# Autodesk Inventor assembly: ASY PRS 2 Filter column D1200 940
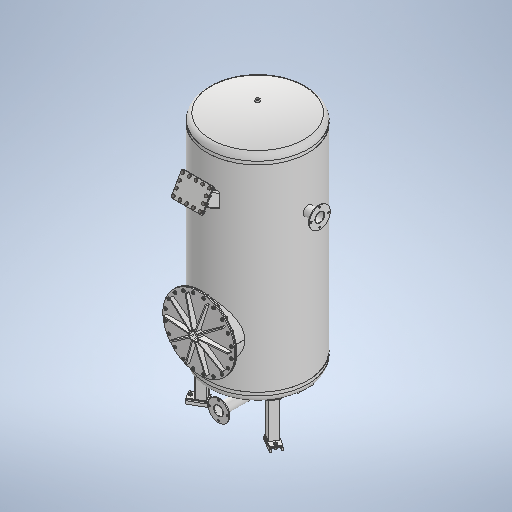
[picture p0: Inventor's stored thumbnail of the model, 512x512]
Saved by Autodesk Inventor 2026.2 (Build 302298000, 298)
## iProperties
Created: 2025-02-13
Part Number: ASY PRS 2 Filter column D1200 940
Document SubType Name: Assembly
Designer: admin
Mass: 296006 g
Surface Area: 199460 cm^2
Volume: 66339.5 cm^3
Density: 4.46198 g/cm^3
Author: pokla
Revision Number: 3
## Documents named in this file (27)
- C:\Users\admin\Documents\Inventor\PRS-Purovsk\ASY PRS 2 Filter column D1200 940.iam
- C:\Users\admin\Documents\Inventor\PRS-Purovsk\PRS 0101 main shell D1200.ipt
- C:\Users\admin\Documents\Inventor\PRS-Purovsk\PRS 0101 main shell D1200 940.ipt
- C:\Users\admin\Documents\Inventor\PRS-Purovsk\PRS 1604 dished head_D1200 940.ipt
- C:\Users\admin\Documents\Inventor\PRS-Purovsk\Fitting G1_D1200 940.ipt
- C:\Users\admin\Documents\Inventor\PRS-Purovsk\PRS 1633 charging blind flange_D1200 940.ipt
- C:\Users\admin\Documents\Inventor\PRS-Purovsk\PRS 8123 pallet jack dummy_D1200.ipt
- C:\Users\admin\Documents\Inventor\PRS-Purovsk\ASY PRS 1610 charging hatch_D1200 940.iam
- C:\Users\admin\Documents\Inventor\PRS-Purovsk\PRS 9612 accses hatch flangeipt_D1200 940.ipt
- C:\Users\admin\Documents\Inventor\PRS-Purovsk\PRS 9607 charging flange rect_D1200 940.ipt
- C:\Users\admin\Documents\Inventor\PRS-Purovsk\PRS 9606 charging flange round_D1200 940.ipt
- C:\Users\admin\Documents\Inventor\PRS-Purovsk\PRS 9672 charging tube 2_D1200 940.ipt
- C:\Users\admin\Documents\Inventor\PRS-Purovsk\PRS 9615 FDS tube 5_D1200 940.ipt
- C:\Users\admin\Documents\Inventor\PRS-Purovsk\PRS 9612 FDS tube 2_D1200 940.ipt
- C:\Users\admin\Documents\Inventor\PRS-Purovsk\cc\JIS B 2312 90 Deg Long Elbow Steel 80A x Sch 40.ipt
- C:\Users\admin\Documents\Inventor\PRS-Purovsk\PRS 9311 accses hatch tube_D1200 940.ipt
- C:\Users\admin\Documents\Inventor\PRS-Purovsk\PRS 9432 FDS free flange DN90_D1200 940.ipt
- C:\Users\admin\Documents\Inventor\PRS-Purovsk\PRS 9431 FDS flange DN90_D1200 940.ipt
- C:\Users\admin\Documents\Inventor\PRS-Purovsk\PRS 9614 FDS tube 4_D1200 940.ipt
- C:\Users\admin\Documents\Inventor\PRS-Purovsk\PRS 9613 FDS tube 3_D1200 940.ipt
- C:\Users\admin\Documents\Inventor\PRS-Purovsk\ASY PRS 9690 Filter legs D1200 940.iam
- C:\Users\admin\Documents\Inventor\PRS-Purovsk\cc\en-US\ISO 4018\ISO 4018 - M16 x 40.ipt
- C:\Users\admin\Documents\Inventor\PRS-Purovsk\cc\en-US\ISO 7089\ISO 7089 - 16 - 140 HV(1).ipt
- C:\Users\admin\Documents\Inventor\PRS-Purovsk\cc\en-US\ISO 4032(2)\ISO 4032 - M16 - ISO.ipt
- C:\Users\admin\Documents\Inventor\PRS-Purovsk\cc\en-US\ISO 4017(1)\ISO 4017 - M16 x 35 - ISO.ipt
- C:\Users\admin\Documents\Inventor\PRS-Purovsk\cc\en-US\ISO 7090\ISO 7090 - 16 - 140 HV(1).ipt
- C:\Users\admin\Documents\Inventor\PRS-Purovsk\cc\en-US\ISO 4033(2)\ISO 4033 - M16 - ISO.ipt
## Components (127 placed, 25 different names)
1. PRS 0101 main shell D1200 940:1 — Mate:1, Flush:4, Flush:2, Tangent:1, Mate:10, Mate:9, Rigid:16, Rotational:2, Rotational:3
2. PRS 1604 dished head_D1200 940:1 — Mate:8, Rigid:20, Mate:5, Mate:147, Mate:148, Rotational:2
3. PRS 1604 dished head_D1200 940:2 — Mate:4, Rigid:15, Rotational:3
4. Fitting G1_D1200 940:1 — Rigid:15
5. PRS 1633 charging blind flange_D1200 940:1 — Rigid:67
6. PRS 8123 pallet jack dummy_D1200:1
7. PRS 1633 charging blind flange_D1200 940:2 — Rigid:18
8. PRS 1633 charging blind flange_D1200 940:3 — Rigid:78
9. ASY PRS 1610 charging hatch_D1200 940:1 [sub-assembly] — Mate:12, Mate:11, Mate:51, Mate:14, Mate:13, Mate:16, Mate:15, Mate:18, Mate:17, Mate:20, Mate:19, Mate:22, Mate:21, Mate:24, Mate:23, Mate:26, Mate:25, Mate:28, Mate:27, Mate:30, Mate:29, Mate:32, Mate:31, Mate:34, Mate:33, Mate:36, Mate:35, Mate:38, Mate:37, Mate:40, Mate:39, Mate:42, Mate:41, Mate:44, Mate:43, Mate:46, Mate:45, Mate:48, Mate:47, Mate:50, Mate:49, Mate:53, Mate:55, Mate:57, Mate:59, Mate:61, Mate:63, Mate:65, Mate:67, Mate:69, Mate:71, Mate:73, Mate:75, Mate:77, Mate:79, Mate:81, Mate:83, Mate:85, Mate:87, Mate:89, Rigid:24
10. PRS 9612 accses hatch flangeipt_D1200 940:1 — Mate:52, Mate:54, Mate:56, Mate:58, Mate:60, Mate:62, Mate:64, Mate:66, Mate:68, Mate:70, Mate:72, Mate:74, Mate:76, Mate:78, Mate:80, Mate:82, Mate:84, Mate:86, Mate:88, Mate:90, Rigid:24, Rigid:23
11. PRS 9607 charging flange rect_D1200 940:1 — Mate:92, Mate:91, Mate:119, Mate:94, Mate:93, Mate:96, Mate:95, Mate:98, Mate:97, Mate:100, Mate:99, Mate:102, Mate:101, Mate:104, Mate:103, Mate:106, Mate:105, Mate:108, Mate:107, Mate:110, Mate:109, Mate:112, Mate:111, Mate:114, Mate:113, Mate:116, Mate:115, Mate:118, Mate:117, Mate:121, Mate:123, Mate:125, Mate:127, Mate:129, Mate:131, Mate:133, Mate:135, Mate:137, Mate:139, Mate:141, Mate:143, Mate:145, Rigid:83
12. PRS 9606 charging flange round_D1200 940:1 — Tangent:1, Mate:120, Mate:122, Mate:124, Mate:126, Mate:128, Mate:130, Mate:132, Mate:134, Mate:136, Mate:138, Mate:140, Mate:142, Mate:144, Mate:146, Rigid:83, Rigid:22
13. PRS 9672 charging tube 2_D1200 940:1 — Mate:10, Mate:9, Rigid:21
14. PRS 9615 FDS tube 5_D1200 940:1 — Rigid:17, Rigid:18
15. PRS 9612 FDS tube 2_D1200 940:1 — Mate:4, Rigid:78, Rigid:62
16. JIS B 2312 90 Deg Long Elbow Steel 80A x Sch 40:1 — Rigid:62, Rigid:17
17. PRS 9311 accses hatch tube_D1200 940:1 — Rigid:23, Rigid:16
18. PRS 9432 FDS free flange DN90_D1200 940:1 — Rigid:76, Rotational:71
19. PRS 9431 FDS flange DN90_D1200 940:1 — Rigid:76
20. PRS 9614 FDS tube 4_D1200 940:1 — Rigid:20, Rotational:71, Rigid:79
21. PRS 9613 FDS tube 3_D1200 940:1 — Rigid:67, Rigid:68
22. JIS B 2312 90 Deg Long Elbow Steel 80A x Sch 40:2 — Rigid:79, Rigid:68
23. Fitting G1_D1200 940:2 — Mate:8, Mate:7, Mate:6
24. ASY PRS 9690 Filter legs D1200 940:1 [sub-assembly] — Mate:2, Flush:6, Flush:5
25. PRS 9672 charging tube 2_D1200 940:2 — Rigid:22, Rigid:21
26. ISO 4018 M16 x 40:1 — Mate:12, Mate:11
27. ISO 7089 16:1 — Mate:52, Mate:51, Insert:1
28. ISO 4032 M16:1 — Insert:1
29. ISO 4018 M16 x 40:2 — Mate:14, Mate:13
30. ISO 4018 M16 x 40:3 — Mate:16, Mate:15
31. ISO 4018 M16 x 40:4 — Mate:18, Mate:17
32. ISO 4018 M16 x 40:5 — Mate:20, Mate:19
33. ISO 4018 M16 x 40:6 — Mate:22, Mate:21
34. ISO 4018 M16 x 40:7 — Mate:24, Mate:23
35. ISO 4018 M16 x 40:8 — Mate:26, Mate:25
36. ISO 4018 M16 x 40:9 — Mate:28, Mate:27
37. ISO 4018 M16 x 40:10 — Mate:30, Mate:29
38. ISO 4018 M16 x 40:11 — Mate:32, Mate:31
39. ISO 4018 M16 x 40:12 — Mate:34, Mate:33
40. ISO 4018 M16 x 40:13 — Mate:36, Mate:35
41. ISO 4018 M16 x 40:14 — Mate:38, Mate:37
42. ISO 4018 M16 x 40:15 — Mate:40, Mate:39
43. ISO 4018 M16 x 40:16 — Mate:42, Mate:41
44. ISO 4018 M16 x 40:17 — Mate:44, Mate:43
45. ISO 4018 M16 x 40:18 — Mate:46, Mate:45
46. ISO 4018 M16 x 40:19 — Mate:48, Mate:47
47. ISO 4018 M16 x 40:20 — Mate:50, Mate:49
48. ISO 7089 16:2 — Mate:54, Mate:53, Insert:2
49. ISO 7089 16:3 — Mate:56, Mate:55, Insert:3
50. ISO 7089 16:4 — Mate:58, Mate:57, Insert:4
51. ISO 7089 16:5 — Mate:60, Mate:59, Insert:5
52. ISO 7089 16:6 — Mate:62, Mate:61, Insert:6
53. ISO 7089 16:7 — Mate:64, Mate:63, Insert:7
54. ISO 7089 16:8 — Mate:66, Mate:65, Insert:8
55. ISO 7089 16:9 — Mate:68, Mate:67, Insert:9
56. ISO 7089 16:10 — Mate:70, Mate:69, Insert:10
57. ISO 7089 16:11 — Mate:72, Mate:71, Insert:11
58. ISO 7089 16:12 — Mate:74, Mate:73, Insert:12
59. ISO 7089 16:13 — Mate:76, Mate:75, Insert:13
60. ISO 7089 16:14 — Mate:78, Mate:77, Insert:14
61. ISO 7089 16:15 — Mate:80, Mate:79, Insert:15
62. ISO 7089 16:16 — Mate:82, Mate:81, Insert:16
63. ISO 7089 16:17 — Mate:84, Mate:83, Insert:17
64. ISO 7089 16:18 — Mate:86, Mate:85, Insert:18
65. ISO 7089 16:19 — Mate:88, Mate:87, Insert:19
66. ISO 7089 16:20 — Mate:90, Mate:89, Insert:20
67. ISO 4032 M16:2 — Insert:2
68. ISO 4032 M16:3 — Insert:3
69. ISO 4032 M16:4 — Insert:4
70. ISO 4032 M16:5 — Insert:5
71. ISO 4032 M16:6 — Insert:6
72. ISO 4032 M16:7 — Insert:7
73. ISO 4032 M16:8 — Insert:8
74. ISO 4032 M16:9 — Insert:9
75. ISO 4032 M16:10 — Insert:10
76. ISO 4032 M16:11 — Insert:11
77. ISO 4032 M16:12 — Insert:12
78. ISO 4032 M16:13 — Insert:13
79. ISO 4032 M16:14 — Insert:14
80. ISO 4032 M16:15 — Insert:15
81. ISO 4032 M16:16 — Insert:16
82. ISO 4032 M16:17 — Insert:17
83. ISO 4032 M16:18 — Insert:18
84. ISO 4032 M16:19 — Insert:19
85. ISO 4032 M16:20 — Insert:20
86. ISO 4017 M16 x 35:1 — Mate:92, Mate:91
87. ISO 7090 16 - 140 HV:1 — Mate:120, Mate:119, Insert:21
88. ISO 4033 M16:1 — Insert:21
89. ISO 4017 M16 x 35:2 — Mate:94, Mate:93
90. ISO 4017 M16 x 35:3 — Mate:96, Mate:95
91. ISO 4017 M16 x 35:4 — Mate:98, Mate:97
92. ISO 4017 M16 x 35:5 — Mate:100, Mate:99
93. ISO 4017 M16 x 35:6 — Mate:102, Mate:101
94. ISO 4017 M16 x 35:7 — Mate:104, Mate:103
95. ISO 4017 M16 x 35:8 — Mate:106, Mate:105
96. ISO 4017 M16 x 35:9 — Mate:108, Mate:107
97. ISO 4017 M16 x 35:10 — Mate:110, Mate:109
98. ISO 4017 M16 x 35:11 — Mate:112, Mate:111
99. ISO 4017 M16 x 35:12 — Mate:114, Mate:113
100. ISO 4017 M16 x 35:13 — Mate:116, Mate:115
101. ISO 4017 M16 x 35:14 — Mate:118, Mate:117
102. ISO 7090 16 - 140 HV:2 — Mate:122, Mate:121, Insert:22
103. ISO 7090 16 - 140 HV:3 — Mate:124, Mate:123, Insert:23
104. ISO 7090 16 - 140 HV:4 — Mate:126, Mate:125, Insert:24
105. ISO 7090 16 - 140 HV:5 — Mate:128, Mate:127, Insert:25
106. ISO 7090 16 - 140 HV:6 — Mate:130, Mate:129, Insert:26
107. ISO 7090 16 - 140 HV:7 — Mate:132, Mate:131, Insert:27
108. ISO 7090 16 - 140 HV:8 — Mate:134, Mate:133, Insert:28
109. ISO 7090 16 - 140 HV:9 — Mate:136, Mate:135, Insert:29
110. ISO 7090 16 - 140 HV:10 — Mate:138, Mate:137, Insert:30
111. ISO 7090 16 - 140 HV:11 — Mate:140, Mate:139, Insert:31
112. ISO 7090 16 - 140 HV:12 — Mate:142, Mate:141, Insert:32
113. ISO 7090 16 - 140 HV:13 — Mate:144, Mate:143, Insert:33
114. ISO 7090 16 - 140 HV:14 — Mate:146, Mate:145, Insert:34
115. ISO 4033 M16:2 — Insert:22
116. ISO 4033 M16:3 — Insert:23
117. ISO 4033 M16:4 — Insert:24
118. ISO 4033 M16:5 — Insert:25
119. ISO 4033 M16:6 — Insert:26
120. ISO 4033 M16:7 — Insert:27
121. ISO 4033 M16:8 — Insert:28
122. ISO 4033 M16:9 — Insert:29
123. ISO 4033 M16:10 — Insert:30
124. ISO 4033 M16:11 — Insert:31
125. ISO 4033 M16:12 — Insert:32
126. ISO 4033 M16:13 — Insert:33
127. ISO 4033 M16:14 — Insert:34
## Relationships (205: Mate 147, Insert 34, WeldJoint 16, Flush 4, RevoluteJoint 3, Tangent 1)
- Mate:1: PRS 0101 main shell D1200 940:1
- Flush:4: PRS 0101 main shell D1200 940:1
- Flush:2: PRS 0101 main shell D1200 940:1
- Tangent:1 (80 mm): PRS 0101 main shell D1200 940:1 ↔ PRS 9606 charging flange round_D1200 940:1
- Mate:10: PRS 0101 main shell D1200 940:1 ↔ PRS 9672 charging tube 2_D1200 940:1
- Mate:9: PRS 0101 main shell D1200 940:1 ↔ PRS 9672 charging tube 2_D1200 940:1
- Mate:4: PRS 1604 dished head_D1200 940:2 ↔ PRS 9612 FDS tube 2_D1200 940:1
- Mate:8: PRS 1604 dished head_D1200 940:1 ↔ Fitting G1_D1200 940:2
- Mate:7 (150 mm): Fitting G1_D1200 940:2
- Mate:6: Fitting G1_D1200 940:2
- Mate:2: ASY PRS 9690 Filter legs D1200 940:1
- Flush:6: ASY PRS 9690 Filter legs D1200 940:1
- Flush:5: ASY PRS 9690 Filter legs D1200 940:1
- Mate:12: ASY PRS 1610 charging hatch_D1200 940:1 ↔ ISO 4018 M16 x 40:1
- Mate:11: ASY PRS 1610 charging hatch_D1200 940:1 ↔ ISO 4018 M16 x 40:1
- Mate:52: PRS 9612 accses hatch flangeipt_D1200 940:1 ↔ ISO 7089 16:1
- Mate:51: ASY PRS 1610 charging hatch_D1200 940:1 ↔ ISO 7089 16:1
- Insert:1: ISO 7089 16:1 ↔ ISO 4032 M16:1
- Mate:14: ASY PRS 1610 charging hatch_D1200 940:1 ↔ ISO 4018 M16 x 40:2
- Mate:13: ASY PRS 1610 charging hatch_D1200 940:1 ↔ ISO 4018 M16 x 40:2
- Mate:16: ASY PRS 1610 charging hatch_D1200 940:1 ↔ ISO 4018 M16 x 40:3
- Mate:15: ASY PRS 1610 charging hatch_D1200 940:1 ↔ ISO 4018 M16 x 40:3
- Mate:18: ASY PRS 1610 charging hatch_D1200 940:1 ↔ ISO 4018 M16 x 40:4
- Mate:17: ASY PRS 1610 charging hatch_D1200 940:1 ↔ ISO 4018 M16 x 40:4
- Mate:20: ASY PRS 1610 charging hatch_D1200 940:1 ↔ ISO 4018 M16 x 40:5
- Mate:19: ASY PRS 1610 charging hatch_D1200 940:1 ↔ ISO 4018 M16 x 40:5
- Mate:22: ASY PRS 1610 charging hatch_D1200 940:1 ↔ ISO 4018 M16 x 40:6
- Mate:21: ASY PRS 1610 charging hatch_D1200 940:1 ↔ ISO 4018 M16 x 40:6
- Mate:24: ASY PRS 1610 charging hatch_D1200 940:1 ↔ ISO 4018 M16 x 40:7
- Mate:23: ASY PRS 1610 charging hatch_D1200 940:1 ↔ ISO 4018 M16 x 40:7
- Mate:26: ASY PRS 1610 charging hatch_D1200 940:1 ↔ ISO 4018 M16 x 40:8
- Mate:25: ASY PRS 1610 charging hatch_D1200 940:1 ↔ ISO 4018 M16 x 40:8
- Mate:28: ASY PRS 1610 charging hatch_D1200 940:1 ↔ ISO 4018 M16 x 40:9
- Mate:27: ASY PRS 1610 charging hatch_D1200 940:1 ↔ ISO 4018 M16 x 40:9
- Mate:30: ASY PRS 1610 charging hatch_D1200 940:1 ↔ ISO 4018 M16 x 40:10
- Mate:29: ASY PRS 1610 charging hatch_D1200 940:1 ↔ ISO 4018 M16 x 40:10
- Mate:32: ASY PRS 1610 charging hatch_D1200 940:1 ↔ ISO 4018 M16 x 40:11
- Mate:31: ASY PRS 1610 charging hatch_D1200 940:1 ↔ ISO 4018 M16 x 40:11
- Mate:34: ASY PRS 1610 charging hatch_D1200 940:1 ↔ ISO 4018 M16 x 40:12
- Mate:33: ASY PRS 1610 charging hatch_D1200 940:1 ↔ ISO 4018 M16 x 40:12
- Mate:36: ASY PRS 1610 charging hatch_D1200 940:1 ↔ ISO 4018 M16 x 40:13
- Mate:35: ASY PRS 1610 charging hatch_D1200 940:1 ↔ ISO 4018 M16 x 40:13
- Mate:38: ASY PRS 1610 charging hatch_D1200 940:1 ↔ ISO 4018 M16 x 40:14
- Mate:37: ASY PRS 1610 charging hatch_D1200 940:1 ↔ ISO 4018 M16 x 40:14
- Mate:40: ASY PRS 1610 charging hatch_D1200 940:1 ↔ ISO 4018 M16 x 40:15
- Mate:39: ASY PRS 1610 charging hatch_D1200 940:1 ↔ ISO 4018 M16 x 40:15
- Mate:42: ASY PRS 1610 charging hatch_D1200 940:1 ↔ ISO 4018 M16 x 40:16
- Mate:41: ASY PRS 1610 charging hatch_D1200 940:1 ↔ ISO 4018 M16 x 40:16
- Mate:44: ASY PRS 1610 charging hatch_D1200 940:1 ↔ ISO 4018 M16 x 40:17
- Mate:43: ASY PRS 1610 charging hatch_D1200 940:1 ↔ ISO 4018 M16 x 40:17
- Mate:46: ASY PRS 1610 charging hatch_D1200 940:1 ↔ ISO 4018 M16 x 40:18
- Mate:45: ASY PRS 1610 charging hatch_D1200 940:1 ↔ ISO 4018 M16 x 40:18
- Mate:48: ASY PRS 1610 charging hatch_D1200 940:1 ↔ ISO 4018 M16 x 40:19
- Mate:47: ASY PRS 1610 charging hatch_D1200 940:1 ↔ ISO 4018 M16 x 40:19
- Mate:50: ASY PRS 1610 charging hatch_D1200 940:1 ↔ ISO 4018 M16 x 40:20
- Mate:49: ASY PRS 1610 charging hatch_D1200 940:1 ↔ ISO 4018 M16 x 40:20
- Mate:54: PRS 9612 accses hatch flangeipt_D1200 940:1 ↔ ISO 7089 16:2
- Mate:53: ASY PRS 1610 charging hatch_D1200 940:1 ↔ ISO 7089 16:2
- Mate:56: PRS 9612 accses hatch flangeipt_D1200 940:1 ↔ ISO 7089 16:3
- Mate:55: ASY PRS 1610 charging hatch_D1200 940:1 ↔ ISO 7089 16:3
- Mate:58: PRS 9612 accses hatch flangeipt_D1200 940:1 ↔ ISO 7089 16:4
- Mate:57: ASY PRS 1610 charging hatch_D1200 940:1 ↔ ISO 7089 16:4
- Mate:60: PRS 9612 accses hatch flangeipt_D1200 940:1 ↔ ISO 7089 16:5
- Mate:59: ASY PRS 1610 charging hatch_D1200 940:1 ↔ ISO 7089 16:5
- Mate:62: PRS 9612 accses hatch flangeipt_D1200 940:1 ↔ ISO 7089 16:6
- Mate:61: ASY PRS 1610 charging hatch_D1200 940:1 ↔ ISO 7089 16:6
- Mate:64: PRS 9612 accses hatch flangeipt_D1200 940:1 ↔ ISO 7089 16:7
- Mate:63: ASY PRS 1610 charging hatch_D1200 940:1 ↔ ISO 7089 16:7
- Mate:66: PRS 9612 accses hatch flangeipt_D1200 940:1 ↔ ISO 7089 16:8
- Mate:65: ASY PRS 1610 charging hatch_D1200 940:1 ↔ ISO 7089 16:8
- Mate:68: PRS 9612 accses hatch flangeipt_D1200 940:1 ↔ ISO 7089 16:9
- Mate:67: ASY PRS 1610 charging hatch_D1200 940:1 ↔ ISO 7089 16:9
- Mate:70: PRS 9612 accses hatch flangeipt_D1200 940:1 ↔ ISO 7089 16:10
- Mate:69: ASY PRS 1610 charging hatch_D1200 940:1 ↔ ISO 7089 16:10
- Mate:72: PRS 9612 accses hatch flangeipt_D1200 940:1 ↔ ISO 7089 16:11
- Mate:71: ASY PRS 1610 charging hatch_D1200 940:1 ↔ ISO 7089 16:11
- Mate:74: PRS 9612 accses hatch flangeipt_D1200 940:1 ↔ ISO 7089 16:12
- Mate:73: ASY PRS 1610 charging hatch_D1200 940:1 ↔ ISO 7089 16:12
- Mate:76: PRS 9612 accses hatch flangeipt_D1200 940:1 ↔ ISO 7089 16:13
- Mate:75: ASY PRS 1610 charging hatch_D1200 940:1 ↔ ISO 7089 16:13
- Mate:78: PRS 9612 accses hatch flangeipt_D1200 940:1 ↔ ISO 7089 16:14
- Mate:77: ASY PRS 1610 charging hatch_D1200 940:1 ↔ ISO 7089 16:14
- Mate:80: PRS 9612 accses hatch flangeipt_D1200 940:1 ↔ ISO 7089 16:15
- Mate:79: ASY PRS 1610 charging hatch_D1200 940:1 ↔ ISO 7089 16:15
- Mate:82: PRS 9612 accses hatch flangeipt_D1200 940:1 ↔ ISO 7089 16:16
- Mate:81: ASY PRS 1610 charging hatch_D1200 940:1 ↔ ISO 7089 16:16
- Mate:84: PRS 9612 accses hatch flangeipt_D1200 940:1 ↔ ISO 7089 16:17
- Mate:83: ASY PRS 1610 charging hatch_D1200 940:1 ↔ ISO 7089 16:17
- Mate:86: PRS 9612 accses hatch flangeipt_D1200 940:1 ↔ ISO 7089 16:18
- Mate:85: ASY PRS 1610 charging hatch_D1200 940:1 ↔ ISO 7089 16:18
- Mate:88: PRS 9612 accses hatch flangeipt_D1200 940:1 ↔ ISO 7089 16:19
- Mate:87: ASY PRS 1610 charging hatch_D1200 940:1 ↔ ISO 7089 16:19
- Mate:90: PRS 9612 accses hatch flangeipt_D1200 940:1 ↔ ISO 7089 16:20
- Mate:89: ASY PRS 1610 charging hatch_D1200 940:1 ↔ ISO 7089 16:20
- Insert:2: ISO 7089 16:2 ↔ ISO 4032 M16:2
- Insert:3: ISO 7089 16:3 ↔ ISO 4032 M16:3
- Insert:4: ISO 7089 16:4 ↔ ISO 4032 M16:4
- Insert:5: ISO 7089 16:5 ↔ ISO 4032 M16:5
- Insert:6: ISO 7089 16:6 ↔ ISO 4032 M16:6
- Insert:7: ISO 7089 16:7 ↔ ISO 4032 M16:7
- Insert:8: ISO 7089 16:8 ↔ ISO 4032 M16:8
- Insert:9: ISO 7089 16:9 ↔ ISO 4032 M16:9
- Insert:10: ISO 7089 16:10 ↔ ISO 4032 M16:10
- Insert:11: ISO 7089 16:11 ↔ ISO 4032 M16:11
- Insert:12: ISO 7089 16:12 ↔ ISO 4032 M16:12
- Insert:13: ISO 7089 16:13 ↔ ISO 4032 M16:13
- Insert:14: ISO 7089 16:14 ↔ ISO 4032 M16:14
- Insert:15: ISO 7089 16:15 ↔ ISO 4032 M16:15
- Insert:16: ISO 7089 16:16 ↔ ISO 4032 M16:16
- Insert:17: ISO 7089 16:17 ↔ ISO 4032 M16:17
- Insert:18: ISO 7089 16:18 ↔ ISO 4032 M16:18
- Insert:19: ISO 7089 16:19 ↔ ISO 4032 M16:19
- Insert:20: ISO 7089 16:20 ↔ ISO 4032 M16:20
- Mate:92: PRS 9607 charging flange rect_D1200 940:1 ↔ ISO 4017 M16 x 35:1
- Mate:91: PRS 9607 charging flange rect_D1200 940:1 ↔ ISO 4017 M16 x 35:1
- Mate:120: PRS 9606 charging flange round_D1200 940:1 ↔ ISO 7090 16 - 140 HV:1
- Mate:119: PRS 9607 charging flange rect_D1200 940:1 ↔ ISO 7090 16 - 140 HV:1
- Insert:21: ISO 7090 16 - 140 HV:1 ↔ ISO 4033 M16:1
- Mate:94: PRS 9607 charging flange rect_D1200 940:1 ↔ ISO 4017 M16 x 35:2
- Mate:93: PRS 9607 charging flange rect_D1200 940:1 ↔ ISO 4017 M16 x 35:2
- Mate:96: PRS 9607 charging flange rect_D1200 940:1 ↔ ISO 4017 M16 x 35:3
- Mate:95: PRS 9607 charging flange rect_D1200 940:1 ↔ ISO 4017 M16 x 35:3
- Mate:98: PRS 9607 charging flange rect_D1200 940:1 ↔ ISO 4017 M16 x 35:4
- Mate:97: PRS 9607 charging flange rect_D1200 940:1 ↔ ISO 4017 M16 x 35:4
- Mate:100: PRS 9607 charging flange rect_D1200 940:1 ↔ ISO 4017 M16 x 35:5
- Mate:99: PRS 9607 charging flange rect_D1200 940:1 ↔ ISO 4017 M16 x 35:5
- Mate:102: PRS 9607 charging flange rect_D1200 940:1 ↔ ISO 4017 M16 x 35:6
- Mate:101: PRS 9607 charging flange rect_D1200 940:1 ↔ ISO 4017 M16 x 35:6
- Mate:104: PRS 9607 charging flange rect_D1200 940:1 ↔ ISO 4017 M16 x 35:7
- Mate:103: PRS 9607 charging flange rect_D1200 940:1 ↔ ISO 4017 M16 x 35:7
- Mate:106: PRS 9607 charging flange rect_D1200 940:1 ↔ ISO 4017 M16 x 35:8
- Mate:105: PRS 9607 charging flange rect_D1200 940:1 ↔ ISO 4017 M16 x 35:8
- Mate:108: PRS 9607 charging flange rect_D1200 940:1 ↔ ISO 4017 M16 x 35:9
- Mate:107: PRS 9607 charging flange rect_D1200 940:1 ↔ ISO 4017 M16 x 35:9
- Mate:110: PRS 9607 charging flange rect_D1200 940:1 ↔ ISO 4017 M16 x 35:10
- Mate:109: PRS 9607 charging flange rect_D1200 940:1 ↔ ISO 4017 M16 x 35:10
- Mate:112: PRS 9607 charging flange rect_D1200 940:1 ↔ ISO 4017 M16 x 35:11
- Mate:111: PRS 9607 charging flange rect_D1200 940:1 ↔ ISO 4017 M16 x 35:11
- Mate:114: PRS 9607 charging flange rect_D1200 940:1 ↔ ISO 4017 M16 x 35:12
- Mate:113: PRS 9607 charging flange rect_D1200 940:1 ↔ ISO 4017 M16 x 35:12
- Mate:116: PRS 9607 charging flange rect_D1200 940:1 ↔ ISO 4017 M16 x 35:13
- Mate:115: PRS 9607 charging flange rect_D1200 940:1 ↔ ISO 4017 M16 x 35:13
- Mate:118: PRS 9607 charging flange rect_D1200 940:1 ↔ ISO 4017 M16 x 35:14
- Mate:117: PRS 9607 charging flange rect_D1200 940:1 ↔ ISO 4017 M16 x 35:14
- Mate:122: PRS 9606 charging flange round_D1200 940:1 ↔ ISO 7090 16 - 140 HV:2
- Mate:121: PRS 9607 charging flange rect_D1200 940:1 ↔ ISO 7090 16 - 140 HV:2
- Mate:124: PRS 9606 charging flange round_D1200 940:1 ↔ ISO 7090 16 - 140 HV:3
- Mate:123: PRS 9607 charging flange rect_D1200 940:1 ↔ ISO 7090 16 - 140 HV:3
- Mate:126: PRS 9606 charging flange round_D1200 940:1 ↔ ISO 7090 16 - 140 HV:4
- Mate:125: PRS 9607 charging flange rect_D1200 940:1 ↔ ISO 7090 16 - 140 HV:4
- Mate:128: PRS 9606 charging flange round_D1200 940:1 ↔ ISO 7090 16 - 140 HV:5
- Mate:127: PRS 9607 charging flange rect_D1200 940:1 ↔ ISO 7090 16 - 140 HV:5
- Mate:130: PRS 9606 charging flange round_D1200 940:1 ↔ ISO 7090 16 - 140 HV:6
- Mate:129: PRS 9607 charging flange rect_D1200 940:1 ↔ ISO 7090 16 - 140 HV:6
- Mate:132: PRS 9606 charging flange round_D1200 940:1 ↔ ISO 7090 16 - 140 HV:7
- Mate:131: PRS 9607 charging flange rect_D1200 940:1 ↔ ISO 7090 16 - 140 HV:7
- Mate:134: PRS 9606 charging flange round_D1200 940:1 ↔ ISO 7090 16 - 140 HV:8
- Mate:133: PRS 9607 charging flange rect_D1200 940:1 ↔ ISO 7090 16 - 140 HV:8
- Mate:136: PRS 9606 charging flange round_D1200 940:1 ↔ ISO 7090 16 - 140 HV:9
- Mate:135: PRS 9607 charging flange rect_D1200 940:1 ↔ ISO 7090 16 - 140 HV:9
- Mate:138: PRS 9606 charging flange round_D1200 940:1 ↔ ISO 7090 16 - 140 HV:10
- Mate:137: PRS 9607 charging flange rect_D1200 940:1 ↔ ISO 7090 16 - 140 HV:10
- Mate:140: PRS 9606 charging flange round_D1200 940:1 ↔ ISO 7090 16 - 140 HV:11
- Mate:139: PRS 9607 charging flange rect_D1200 940:1 ↔ ISO 7090 16 - 140 HV:11
- Mate:142: PRS 9606 charging flange round_D1200 940:1 ↔ ISO 7090 16 - 140 HV:12
- Mate:141: PRS 9607 charging flange rect_D1200 940:1 ↔ ISO 7090 16 - 140 HV:12
- Mate:144: PRS 9606 charging flange round_D1200 940:1 ↔ ISO 7090 16 - 140 HV:13
- Mate:143: PRS 9607 charging flange rect_D1200 940:1 ↔ ISO 7090 16 - 140 HV:13
- Mate:146: PRS 9606 charging flange round_D1200 940:1 ↔ ISO 7090 16 - 140 HV:14
- Mate:145: PRS 9607 charging flange rect_D1200 940:1 ↔ ISO 7090 16 - 140 HV:14
- Insert:22: ISO 7090 16 - 140 HV:2 ↔ ISO 4033 M16:2
- Insert:23: ISO 7090 16 - 140 HV:3 ↔ ISO 4033 M16:3
- Insert:24: ISO 7090 16 - 140 HV:4 ↔ ISO 4033 M16:4
- Insert:25: ISO 7090 16 - 140 HV:5 ↔ ISO 4033 M16:5
- Insert:26: ISO 7090 16 - 140 HV:6 ↔ ISO 4033 M16:6
- Insert:27: ISO 7090 16 - 140 HV:7 ↔ ISO 4033 M16:7
- Insert:28: ISO 7090 16 - 140 HV:8 ↔ ISO 4033 M16:8
- Insert:29: ISO 7090 16 - 140 HV:9 ↔ ISO 4033 M16:9
- Insert:30: ISO 7090 16 - 140 HV:10 ↔ ISO 4033 M16:10
- Insert:31: ISO 7090 16 - 140 HV:11 ↔ ISO 4033 M16:11
- Insert:32: ISO 7090 16 - 140 HV:12 ↔ ISO 4033 M16:12
- Insert:33: ISO 7090 16 - 140 HV:13 ↔ ISO 4033 M16:13
- Insert:34: ISO 7090 16 - 140 HV:14 ↔ ISO 4033 M16:14
- Rigid:15 [WeldJoint]: PRS 1604 dished head_D1200 940:2 ↔ Fitting G1_D1200 940:1
- Rigid:24 [WeldJoint]: ASY PRS 1610 charging hatch_D1200 940:1 ↔ PRS 9612 accses hatch flangeipt_D1200 940:1
- Rigid:83 [WeldJoint]: PRS 9607 charging flange rect_D1200 940:1 ↔ PRS 9606 charging flange round_D1200 940:1
- Rigid:78 [WeldJoint]: PRS 1633 charging blind flange_D1200 940:3 ↔ PRS 9612 FDS tube 2_D1200 940:1
- Rigid:62 [WeldJoint]: PRS 9612 FDS tube 2_D1200 940:1 ↔ JIS B 2312 90 Deg Long Elbow Steel 80A x Sch 40:1
- Rigid:23 [WeldJoint]: PRS 9612 accses hatch flangeipt_D1200 940:1 ↔ PRS 9311 accses hatch tube_D1200 940:1
- Rigid:16 [WeldJoint] (20 mm): PRS 0101 main shell D1200 940:1 ↔ PRS 9311 accses hatch tube_D1200 940:1
- Rigid:76 [WeldJoint]: PRS 9432 FDS free flange DN90_D1200 940:1 ↔ PRS 9431 FDS flange DN90_D1200 940:1
- Rigid:20 [WeldJoint]: PRS 1604 dished head_D1200 940:1 ↔ PRS 9614 FDS tube 4_D1200 940:1
- Rotational:71 [RevoluteJoint]: PRS 9432 FDS free flange DN90_D1200 940:1 ↔ PRS 9614 FDS tube 4_D1200 940:1
- Rigid:67 [WeldJoint]: PRS 1633 charging blind flange_D1200 940:1 ↔ PRS 9613 FDS tube 3_D1200 940:1
- Rigid:79 [WeldJoint]: PRS 9614 FDS tube 4_D1200 940:1 ↔ JIS B 2312 90 Deg Long Elbow Steel 80A x Sch 40:2
- Rigid:68 [WeldJoint]: PRS 9613 FDS tube 3_D1200 940:1 ↔ JIS B 2312 90 Deg Long Elbow Steel 80A x Sch 40:2
- Mate:5 (300 mm): PRS 1604 dished head_D1200 940:1
- Rigid:22 [WeldJoint]: PRS 9606 charging flange round_D1200 940:1 ↔ PRS 9672 charging tube 2_D1200 940:2
- Rigid:21 [WeldJoint]: PRS 9672 charging tube 2_D1200 940:1 ↔ PRS 9672 charging tube 2_D1200 940:2
- Mate:147: PRS 1604 dished head_D1200 940:1
- Mate:148: PRS 1604 dished head_D1200 940:1
- Rotational:2 [RevoluteJoint]: PRS 0101 main shell D1200 940:1 ↔ PRS 1604 dished head_D1200 940:1
- Rotational:3 [RevoluteJoint]: PRS 0101 main shell D1200 940:1 ↔ PRS 1604 dished head_D1200 940:2
- Rigid:17 [WeldJoint]: PRS 9615 FDS tube 5_D1200 940:1 ↔ JIS B 2312 90 Deg Long Elbow Steel 80A x Sch 40:1
- Rigid:18 [WeldJoint]: PRS 1633 charging blind flange_D1200 940:2 ↔ PRS 9615 FDS tube 5_D1200 940:1
## Named parameters: AA_MAIN_filter_diam = 1200 mm, AccsessHatch_tube_diameter = 530 mm, ChargingHatch_width = 200 mm, ChargingHatch_hight = 120 mm, AA_MAIN_Filter_Clearance = 300 mm, Legs_Tube_lenght = 377.45004 mm, Legs_Tube_cut_angle = 0.41416, Legs_Upper_plate_lenght = 122.38827 mm, Legs_Tube_dim = 80 mm, Legs_Inner_diam = 895.69544 mm
note: some values were not read from the file. Shown as the stored number, unit unknown: "Legs_Tube_cut_angle".
